# Autodesk Inventor assembly: Cargo Assembly
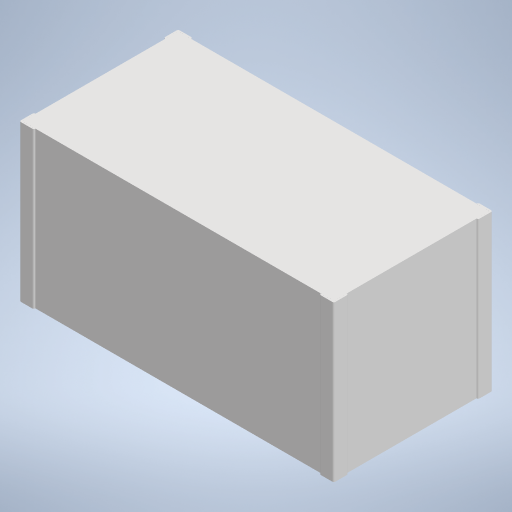
[picture p0: Inventor's stored thumbnail of the model, 512x512]
Saved by Autodesk Inventor 2024.2 (Build 282272000, 272)
## iProperties
Created: 2023-11-13
Part Number: Cargo Assembly
Document SubType Name: Assembly
Designer: Luke
Author: Luke
## Documents named in this file (3)
- C:\Users\Luke\Desktop\Current\Cargo Assembly.iam
- C:\Users\Luke\Desktop\Current\Cargo Container.ipt
- C:\Users\Luke\Desktop\Current\Cargo Aluminum L.ipt
## Components (5 placed, 2 different names)
1. Cargo Container:1 — Mate:1, Mate:2, Mate:3, Mate:4, Mate:5, Mate:6, Mate:7, Mate:8, Mate:9, Mate:10, Mate:11, Mate:12
2. Cargo Aluminum L:1 — Mate:1, Mate:2, Mate:3
3. Cargo Aluminum L:2 — Mate:4, Mate:5, Mate:6
4. Cargo Aluminum L:4 — Mate:7, Mate:8, Mate:9
5. Cargo Aluminum L:5 — Mate:10, Mate:11, Mate:12
## Relationships (12: Mate 12)
- Mate:1: Cargo Container:1 ↔ Cargo Aluminum L:1
- Mate:2: Cargo Container:1 ↔ Cargo Aluminum L:1
- Mate:3: Cargo Container:1 ↔ Cargo Aluminum L:1
- Mate:4: Cargo Container:1 ↔ Cargo Aluminum L:2
- Mate:5: Cargo Container:1 ↔ Cargo Aluminum L:2
- Mate:6: Cargo Container:1 ↔ Cargo Aluminum L:2
- Mate:7: Cargo Container:1 ↔ Cargo Aluminum L:4
- Mate:8: Cargo Container:1 ↔ Cargo Aluminum L:4
- Mate:9: Cargo Container:1 ↔ Cargo Aluminum L:4
- Mate:10: Cargo Container:1 ↔ Cargo Aluminum L:5
- Mate:11: Cargo Container:1 ↔ Cargo Aluminum L:5
- Mate:12: Cargo Container:1 ↔ Cargo Aluminum L:5
